# Autodesk Inventor assembly: Fixture_Plate_Assembly
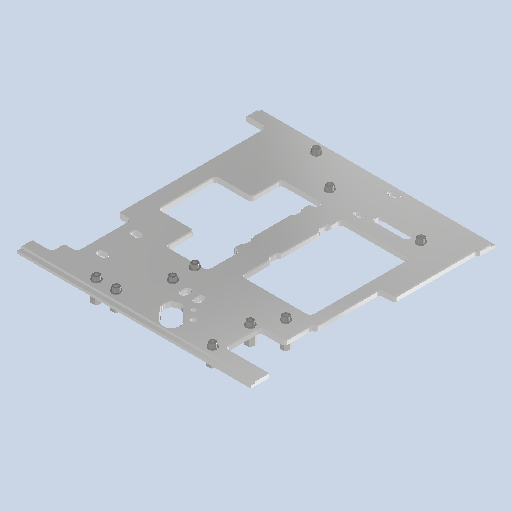
[picture p0: Inventor's stored thumbnail of the model, 512x512]
Saved by Autodesk Inventor 2024.2 (Build 282272000, 272)
## iProperties
Created: 2020-07-14
Part Number: Fixture_Plate_Assembly
Document SubType Name: Assembly
Designer: CASE-SMALL2
Author: CASE-SMALL2
## Documents named in this file (8)
- C:\Users\lgnds\Documents\GitHub\REACH-Hardware\CAD\InventorProject\Fixture_Plate\Fixture_Plate_Assembly.iam
- C:\Users\lgnds\Documents\GitHub\REACH-Hardware\CAD\InventorProject\Fixture_Plate\Fixture_Plate.ipt
- C:\Users\lgnds\Documents\GitHub\REACH-Hardware\CAD\InventorProject\Fixture_Plate\Standsoffs\M2.5x12mm_Standoff_ 970120144.ipt
- C:\Users\lgnds\Documents\GitHub\REACH-Hardware\CAD\InventorProject\Fixture_Plate\Standsoffs\M2.5x9mm_Standoff_ 970090144.ipt
- C:\Users\lgnds\Documents\GitHub\REACH-Hardware\CAD\InventorProject\Fixture_Plate\Standsoffs\M2.5x7mm_Standoff_ 970070151.ipt
- C:\Users\lgnds\Documents\GitHub\REACH-Hardware\CAD\InventorProject\Fixture_Plate\Screws\DIN 125 - A 2.8.ipt
- C:\Users\lgnds\Documents\GitHub\REACH-Hardware\CAD\InventorProject\Fixture_Plate\Screws\ISO 4762 - M2.5 x 8ISO.ipt
- C:\Users\lgnds\Documents\GitHub\REACH-Hardware\CAD\InventorProject\Fixture_Plate\Screws\ISO 4762 - M2.5 x 6ISO.ipt
## Components (31 placed, 7 different names)
1. Fixture_Plate:1 — Rigid:2, Rigid:3, Rigid:5, Rigid:6, Rigid:7, Rigid:8, Rigid:9, Rigid:14, Rigid:15, Rigid:16, Rigid:17, Rigid:18, Rigid:20, Rigid:31, Rigid:32, Rigid:36, Rigid:37, Rigid:33, Rigid:34, Rigid:35
2. M2.5x12mm_Standoff_ 970120144:1 — Rigid:35
3. M2.5x12mm_Standoff_ 970120144:2 — Rigid:3
4. M2.5x12mm_Standoff_ 970120144:3 — Rigid:31
5. M2.5x12mm_Standoff_ 970120144:4 — Rigid:2
6. M2.5x9mm_Standoff_ 970090144:1 — Rigid:7
7. M2.5x9mm_Standoff_ 970090144:2 — Rigid:33
8. M2.5x7mm_Standoff_ 970070151:1 — Rigid:6
9. M2.5x7mm_Standoff_ 970070151:2 — Rigid:5
10. M2.5x7mm_Standoff_ 970070151:3 — Rigid:9
11. M2.5x7mm_Standoff_ 970070151:4 — Rigid:8
12. DIN 125 - A 2.8:1 — Rigid:30, Rigid:37
13. DIN 125 - A 2.8:2 — Rigid:29, Rigid:36
14. DIN 125 - A 2.8:3 — Rigid:28, Rigid:32
15. DIN 125 - A 2.8:4 — Rigid:14, Rigid:22
16. DIN 125 - A 2.8:5 — Rigid:15, Rigid:21
17. DIN 125 - A 2.8:6 — Rigid:27, Rigid:34
18. DIN 125 - A 2.8:7 — Rigid:20, Rigid:25
19. DIN 125 - A 2.8:8 — Rigid:17, Rigid:24
20. DIN 125 - A 2.8:9 — Rigid:18, Rigid:26
21. DIN 125 - A 2.8:10 — Rigid:16, Rigid:23
22. ISO 4762 - M2.5 x 6ISO:1 — Rigid:23
23. ISO 4762 - M2.5 x 6ISO:2 — Rigid:21
24. ISO 4762 - M2.5 x 6ISO:3 — Rigid:24
25. ISO 4762 - M2.5 x 6ISO:4 — Rigid:25
26. ISO 4762 - M2.5 x 8ISO:1 — Rigid:26
27. ISO 4762 - M2.5 x 8ISO:2 — Rigid:27
28. ISO 4762 - M2.5 x 8ISO:3 — Rigid:22
29. ISO 4762 - M2.5 x 8ISO:4 — Rigid:28
30. ISO 4762 - M2.5 x 8ISO:5 — Rigid:29
31. ISO 4762 - M2.5 x 8ISO:6 — Rigid:30
## Relationships (30: WeldJoint 30)
- Rigid:2 [WeldJoint]: Fixture_Plate:1 ↔ M2.5x12mm_Standoff_ 970120144:4
- Rigid:3 [WeldJoint]: Fixture_Plate:1 ↔ M2.5x12mm_Standoff_ 970120144:2
- Rigid:5 [WeldJoint]: Fixture_Plate:1 ↔ M2.5x7mm_Standoff_ 970070151:2
- Rigid:6 [WeldJoint]: Fixture_Plate:1 ↔ M2.5x7mm_Standoff_ 970070151:1
- Rigid:7 [WeldJoint]: Fixture_Plate:1 ↔ M2.5x9mm_Standoff_ 970090144:1
- Rigid:8 [WeldJoint]: Fixture_Plate:1 ↔ M2.5x7mm_Standoff_ 970070151:4
- Rigid:9 [WeldJoint]: Fixture_Plate:1 ↔ M2.5x7mm_Standoff_ 970070151:3
- Rigid:14 [WeldJoint]: Fixture_Plate:1 ↔ DIN 125 - A 2.8:4
- Rigid:15 [WeldJoint]: Fixture_Plate:1 ↔ DIN 125 - A 2.8:5
- Rigid:16 [WeldJoint]: Fixture_Plate:1 ↔ DIN 125 - A 2.8:10
- Rigid:17 [WeldJoint]: Fixture_Plate:1 ↔ DIN 125 - A 2.8:8
- Rigid:18 [WeldJoint]: Fixture_Plate:1 ↔ DIN 125 - A 2.8:9
- Rigid:20 [WeldJoint]: Fixture_Plate:1 ↔ DIN 125 - A 2.8:7
- Rigid:21 [WeldJoint]: DIN 125 - A 2.8:5 ↔ ISO 4762 - M2.5 x 6ISO:2
- Rigid:22 [WeldJoint]: DIN 125 - A 2.8:4 ↔ ISO 4762 - M2.5 x 8ISO:3
- Rigid:23 [WeldJoint]: DIN 125 - A 2.8:10 ↔ ISO 4762 - M2.5 x 6ISO:1
- Rigid:24 [WeldJoint]: DIN 125 - A 2.8:8 ↔ ISO 4762 - M2.5 x 6ISO:3
- Rigid:25 [WeldJoint]: DIN 125 - A 2.8:7 ↔ ISO 4762 - M2.5 x 6ISO:4
- Rigid:26 [WeldJoint]: DIN 125 - A 2.8:9 ↔ ISO 4762 - M2.5 x 8ISO:1
- Rigid:27 [WeldJoint]: DIN 125 - A 2.8:6 ↔ ISO 4762 - M2.5 x 8ISO:2
- Rigid:28 [WeldJoint]: DIN 125 - A 2.8:3 ↔ ISO 4762 - M2.5 x 8ISO:4
- Rigid:29 [WeldJoint]: DIN 125 - A 2.8:2 ↔ ISO 4762 - M2.5 x 8ISO:5
- Rigid:30 [WeldJoint]: DIN 125 - A 2.8:1 ↔ ISO 4762 - M2.5 x 8ISO:6
- Rigid:31 [WeldJoint]: Fixture_Plate:1 ↔ M2.5x12mm_Standoff_ 970120144:3
- Rigid:32 [WeldJoint]: Fixture_Plate:1 ↔ DIN 125 - A 2.8:3
- Rigid:36 [WeldJoint]: Fixture_Plate:1 ↔ DIN 125 - A 2.8:2
- Rigid:37 [WeldJoint]: Fixture_Plate:1 ↔ DIN 125 - A 2.8:1
- Rigid:33 [WeldJoint]: Fixture_Plate:1 ↔ M2.5x9mm_Standoff_ 970090144:2
- Rigid:34 [WeldJoint]: Fixture_Plate:1 ↔ DIN 125 - A 2.8:6
- Rigid:35 [WeldJoint]: Fixture_Plate:1 ↔ M2.5x12mm_Standoff_ 970120144:1
